# Autodesk Inventor assembly: Clutch Concept
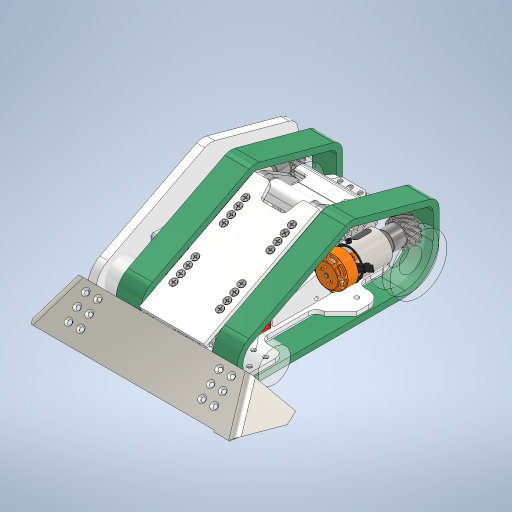
[picture p0: Inventor's stored thumbnail of the model, 512x512]
Saved by Autodesk Inventor 2023.4 (Build 274418000, 418)
## iProperties
Created: 2024-02-03
Part Number: Clutch Concept
Document SubType Name: Assembly
Designer: Nathan Cai
Mass: 1169.62 g
Surface Area: 3186.52 cm^2
Volume: 483.898 cm^3
Density: 2.41709 g/cm^3
Author: Nathan Cai
## Documents named in this file (51)
- E:\Documents\Inventor\Bleep V2\Clutch Concept.iam
- E:\Documents\Inventor\Bleep V2\Flywheel.ipt
- E:\Documents\Inventor\Bleep V2\Thrust Bearing.ipt
- E:\Documents\Inventor\Bleep V2\BB 13x19x4.ipt
- E:\Documents\Inventor\Bleep V2\Cup.ipt
- E:\Documents\Inventor\Bleep V2\1561T741_Stacked Wave Disc Spring\1561T741_Stacked Wave Disc Spring.ipt
- E:\Documents\Inventor\Bleep V2\AKK RS2205 2300KV\AKK RS2205 2300KV.iam
- E:\Documents\Inventor\Bleep V2\Nut Strip 2x1 - 4-40.ipt
- E:\Documents\Inventor\Bleep V2\BB 37mm x 30mm x 4mm.ipt
- E:\Documents\Inventor\Bleep V2\Motor Plate.ipt
- E:\Documents\Inventor\Bleep V2\Uprights.ipt
- E:\Documents\Inventor\Bleep V2\Nut Strip 4x4 - 4-40.ipt
- E:\Documents\Inventor\Bleep V2\5172T23_Metal Gear - 20 Degree Pressure Angle\5172T23_Metal Gear - 20 Degree Pressure Angle.ipt
- E:\Documents\Inventor\Bleep V2\BB .25x.5x.1875 - Flangeless.ipt
- E:\Documents\Inventor\Content Center Files\R2023\en-US\ANSI B18.3(13)\ANSI B18.3 - 4-40 UNC - 0.375(22).ipt
- E:\Documents\Inventor\Bleep V2\Lever.ipt
- E:\Documents\Inventor\Bleep V2\Servo Support.ipt
- E:\Documents\Inventor\Bleep V2\Part1\Part1.ipt
- E:\Documents\Inventor\Bleep V2\Cam - Lever.ipt
- E:\Documents\Inventor\Bleep V2\Cam - Shell.ipt
- E:\Documents\Inventor\Bleep V2\BB 3x7x3.ipt
- E:\Documents\Inventor\Bleep V2\Ramp.ipt
- E:\Documents\Inventor\Bleep V2\Lever - Copy.ipt
- E:\Documents\Inventor\Bleep V2\Brace.ipt
- E:\Documents\Inventor\Bleep V2\BB 3x7x3 - Copy.ipt
- E:\Documents\Inventor\Bleep V2\Shaft - Arms.ipt
- E:\Documents\Inventor\Bleep V2\Shaft - Flywheel C.ipt
- E:\Documents\Inventor\Bleep V2\Clutch C.ipt
- E:\Documents\Inventor\Bleep V2\9293K44_Constant-Force Spring\9293K44_Constant-Force Spring.ipt
- E:\Documents\Inventor\Bleep V2\Spring Mount.ipt
- E:\Documents\Inventor\Bleep V2\Spring Spool.ipt
- E:\Documents\Inventor\Bleep V2\Collar.ipt
- E:\Documents\Inventor\Bleep V2\Bottom Plate.ipt
- E:\Documents\Inventor\Content Center Files\R2023\en-US\ANSI B18.6.3(12)\ANSI B18.6.3 - 4-40 UNC - 0.375(15_).ipt
- E:\Documents\Inventor\Bleep V2\Crown.ipt
- E:\Documents\Inventor\Bleep V2\Front Bumper.ipt
- E:\Documents\Inventor\Content Center Files\R2023\en-US\ANSI B18.6.3(12)\ANSI B18.6.3 - 4-40 UNC - 0.3125(15_).ipt
- E:\Documents\Inventor\Content Center Files\R2023\en-US\ANSI B18.6.3(12)\ANSI B18.6.3 - 6-32 UNC - 0.375(15_).ipt
- E:\Documents\Inventor\Content Center Files\R2023\en-US\ANSI B18.2.2(06)\ANSI B18.2.2 - 6 - 32(06).ipt
- E:\Documents\Inventor\Content Center Files\R2023\en-US\ANSI B18.6.3(14)\ANSI B18.6.3 - 6-32 UNC - 0.625(6).ipt
- E:\Documents\Inventor\Bleep V2\Rack - Slot.ipt
- E:\Documents\Inventor\Bleep V2\Pin Cap - Slot.ipt
- E:\Documents\Inventor\Bleep V2\Export\STL\Lever Spacer.ipt
- E:\Documents\Inventor\Bleep V2\Ranglebox Mars-25 Assembly - Simple\Ranglebox Mars-25 Assembly - Simple.ipt
- E:\Documents\Inventor\Bleep V2\3598N291_High-Power Metal Gear\3598N291_High-Power Metal Gear.ipt
- E:\Documents\Inventor\Bleep V2\Temp Sprocket.ipt
- E:\Documents\Inventor\Bleep V2\Temp Sprocket Front.ipt
- E:\Documents\Inventor\Bleep V2\Temp Tread.ipt
- E:\Documents\Inventor\Bleep V2\Wedge.ipt
- E:\Documents\Inventor\Bleep V2\Temp Side.ipt
- E:\Documents\Inventor\Bleep V2\Tattu 4S 850mah\Tattu 850mah 4S.iam
## Components (124 placed, 50 different names)
1. Front Bumper:1 — Angle:5
2. Bottom Plate:1 — Mate:347, Flush:153, Mate:402, Mate:403, Mate:404, Mate:405, Mate:406, Mate:407, Mate:408, Mate:409, Mate:410, Mate:411, Mate:412, Mate:413, Mate:414, Mate:415, Mate:416, Mate:417, Mate:418, Mate:420, Mate:422, Mate:424, Angle:6
3. Cross Recessed Flat Countersunk Head Machine Screw - Type II - Inch 6-32 x 5/8:1
4. Crown:1 — Mate:386, Mate:387
5. Spline Socket Head Cap Screw - Inch 4-40 UNC - 0.375:9 — Mate:427, Mate:428
6. Spline Socket Head Cap Screw - Inch 4-40 UNC - 0.375:10 — Mate:429, Mate:430
7. Spline Socket Head Cap Screw - Inch 4-40 UNC - 0.375:11 — Mate:431, Mate:432
8. Spline Socket Head Cap Screw - Inch 4-40 UNC - 0.375:12 — Mate:433, Mate:434
9. Spline Socket Head Cap Screw - Inch 4-40 UNC - 0.375:13 — Mate:435, Mate:436
10. Spline Socket Head Cap Screw - Inch 4-40 UNC - 0.375:14 — Mate:437, Mate:438
11. Spline Socket Head Cap Screw - Inch 4-40 UNC - 0.375:15 — Mate:439, Mate:440
12. Spline Socket Head Cap Screw - Inch 4-40 UNC - 0.375:16 — Mate:441, Mate:442
13. Spline Socket Head Cap Screw - Inch 4-40 UNC - 0.375:17 — Mate:443, Mate:444
14. Spline Socket Head Cap Screw - Inch 4-40 UNC - 0.375:18 — Mate:445, Mate:446
15. Spline Socket Head Cap Screw - Inch 4-40 UNC - 0.375:19 — Mate:447, Mate:448
16. Spline Socket Head Cap Screw - Inch 4-40 UNC - 0.375:20 — Mate:449, Mate:450
17. Spline Socket Head Cap Screw - Inch 4-40 UNC - 0.375:21 — Mate:451, Mate:452
18. Spline Socket Head Cap Screw - Inch 4-40 UNC - 0.375:22 — Mate:453, Mate:454
19. Spline Socket Head Cap Screw - Inch 4-40 UNC - 0.375:23 — Mate:455, Mate:456
20. Spline Socket Head Cap Screw - Inch 4-40 UNC - 0.375:24 — Mate:457, Mate:458
21. Pin Cap - Slot:1 — Mate:459, Mate:460, Mate:461
22. Lever Spacer:1 — Mate:462, Mate:463
23. Ranglebox Mars-25 Assembly - Simple:1 — Mate:464, Flush:154, Angle:7
24. 3598N291_High-Power Metal Gear:1 — Mate:464, Flush:154, Tangent:2
25. Temp Sprocket:1 — Tangent:2, Angle:6, Angle:7
26. Temp Sprocket Front:1
27. Temp Tread:1
28. Temp Tread:2
29. Wedge:1
30. Temp Side:1
31. Temp Side:2
32. Ranglebox Mars-25 Assembly - Simple:2
33. 3598N291_High-Power Metal Gear:2
34. Temp Sprocket:2
35. Temp Sprocket Front:2
36. Tattu 850mah 4S:1 [sub-assembly]
37. Flywheel:1 — Mate:275, Mate:309
38. Shaft - Flywheel C:1 — Mate:306, Mate:307, Mate:308, Mate:310, Mate:311, Mate:312, Mate:313, Mate:314, Mate:315, Angle:4, Mate:319, Mate:321, Mate:324, Mate:465
39. Shaft - Arms:1 — Mate:257, Flush:118, Mate:386
40. Clutch C:1 — Mate:308, Angle:4
41. Rack - Slot:1 — Angle:1, Angle:3, Rotation/Translation:1, Mate:315, Mate:313, Mate:314, Mate:459, Mate:460, Mate:461
42. Cup:1 — Mate:26, Mate:27, Angle:1, Tangent:1
43. AKK RS2205 2300KV:1 [sub-assembly] — Mate:426
44. Motor Plate:1 — Mate:106, Mate:107, Mate:128, Mate:129, Mate:131, Mate:132, Mate:134, Mate:136, Flush:106, Mate:144, Mate:145, Mate:146, Mate:147, Mate:148, Mate:149, Mate:150, Mate:151, Mate:152, Mate:153, Mate:154, Mate:155, Mate:156, Mate:157, Mate:158, Mate:159, Flush:149, Mate:426
45. 1561T741_Stacked Wave Disc Spring:1 — Mate:311, Mate:312
46. 9293K44_Constant-Force Spring:1 — Mate:323, Mate:346
47. Spring Mount:1 — Mate:316, Flush:149, Mate:317, Mate:320, Mate:323, Mate:346, Mate:465
48. Thrust Bearing:1 — Mate:319, Mate:320, Mate:322
49. Spring Spool:1 — Mate:321, Mate:322, Mate:325
50. Collar:1 — Mate:324, Mate:325
51. Uprights:1 — Mate:128, Mate:130, Flush:103, Flush:104, Mate:133, Mate:138, Mate:141, Flush:107, Mate:168, Mate:169, Flush:108, Mate:229, Mate:230, Flush:110, Mate:257, Mate:266, Mate:267, Mate:268, Mate:269, Flush:125, Mate:317, Mate:289, Mate:347, Mate:363
52. Uprights:2 — Flush:103, Mate:132, Flush:104, Mate:135, Mate:137, Mate:139, Mate:140, Mate:191, Mate:226, Mate:228, Flush:111, Mate:263, Mate:264, Mate:270, Mate:271, Flush:124, Mate:292, Mate:362, Mate:387, Angle:5
53. Brace:1 — Mate:226, Mate:228, Flush:111, Mate:292
54. Brace:2 — Mate:229, Mate:230, Flush:110, Mate:289
55. Nut Strip 4x4 - 4-40:1 — Mate:129, Mate:130, Mate:131, Mate:133, Mate:316
56. Nut Strip 4x4 - 4-40:2 — Mate:134, Mate:135, Mate:136, Mate:137
57. 5172T23_Metal Gear - 20 Degree Pressure Angle:1 — Mate:138, Mate:141, Flush:105, Angle:3, Mate:198, Mate:199, Mate:200, Mate:201, Mate:202, Mate:203, Mate:204, Rotation/Translation:1, Flush:118, Mate:369, Mate:427, Mate:428, Mate:429, Mate:430, Mate:431, Mate:432, Mate:433, Mate:434, Mate:435, Mate:436, Mate:437, Mate:438, Mate:439, Mate:440, Mate:441, Mate:442
58. 5172T23_Metal Gear - 20 Degree Pressure Angle:2 — Mate:139, Mate:140, Flush:105, Mate:192, Mate:193, Mate:194, Mate:195, Mate:196, Mate:197, Flush:150, Mate:443, Mate:444, Mate:445, Mate:446, Mate:447, Mate:448, Mate:449, Mate:450, Mate:451, Mate:452, Mate:453, Mate:454, Mate:455, Mate:456, Mate:457, Mate:458
59. BB .25x.5x.1875 - Flangeless:1 — Flush:106, Mate:310
60. Lever:1 — Mate:168, Mate:169, Tangent:1, Mate:181, Mate:182, Mate:190, Mate:326, Mate:327
61. Lever - Copy:1
62. Part1:1 — Mate:179, Mate:180, Mate:186, Mate:187, Mate:188
63. Cam - Lever:1 — Mate:177, Mate:178, Mate:327
64. Cam - Shell:1 — Mate:177, Mate:178, Mate:179, Mate:180
65. BB 3x7x3:1 — Mate:181, Mate:182
66. BB 3x7x3:2 — Mate:462, Mate:463
67. BB 3x7x3 - Copy:1 — Mate:190, Mate:326
68. BB 13x19x4:1 — Mate:26, Mate:27
69. BB 37mm x 30mm x 4mm:1 — Mate:106, Mate:107
70. BB .25x.5x.1875 - Flangeless:2 — Mate:275, Mate:306, Mate:307, Mate:309
71. Servo Support:1 — Mate:186, Mate:187, Mate:188, Flush:108, Mate:191, Flush:153, Mate:419, Mate:421, Mate:423, Mate:425
72. Ramp:1 — Mate:204, Flush:150, Mate:369, Mate:370, Mate:371, Mate:372, Mate:373, Mate:374, Mate:375, Mate:376, Mate:377, Mate:378, Mate:379, Mate:380, Mate:381, Mate:382, Mate:383, Mate:384, Mate:385
73. Nut Strip 4x4 - 4-40:3 — Mate:192, Mate:193, Mate:194
74. Nut Strip 4x4 - 4-40:5 — Mate:199, Mate:200, Mate:201
75. Nut Strip 4x4 - 4-40:6 — Mate:198, Mate:202, Mate:203
76. Nut Strip 4x4 - 4-40:7 — Mate:195, Mate:196, Mate:197
77. Nut Strip 4x4 - 4-40:8 — Mate:266, Mate:267, Mate:363
78. Nut Strip 4x4 - 4-40:9 — Mate:263, Mate:264, Mate:362
79. Nut Strip 2x1 - 4-40:3 — Mate:270, Mate:271, Flush:124
80. Nut Strip 2x1 - 4-40:4 — Mate:268, Mate:269, Flush:125
81. Cross Recessed Flat Countersunk Head Machine Screw - Type I - Inch 4-40 x 5/16:1 — Mate:402
82. Cross Recessed Flat Countersunk Head Machine Screw - Type I - Inch 4-40 x 5/16:2 — Mate:403
83. Cross Recessed Flat Countersunk Head Machine Screw - Type I - Inch 4-40 x 5/16:3 — Mate:404
84. Cross Recessed Flat Countersunk Head Machine Screw - Type I - Inch 4-40 x 5/16:4 — Mate:405
85. Cross Recessed Flat Countersunk Head Machine Screw - Type I - Inch 4-40 x 5/16:5 — Mate:406
86. Cross Recessed Flat Countersunk Head Machine Screw - Type I - Inch 4-40 x 5/16:6 — Mate:407
87. Cross Recessed Flat Countersunk Head Machine Screw - Type I - Inch 4-40 x 5/16:7 — Mate:408
88. Cross Recessed Flat Countersunk Head Machine Screw - Type I - Inch 4-40 x 5/16:8 — Mate:409
89. Cross Recessed Flat Countersunk Head Machine Screw - Type I - Inch 4-40 x 5/16:9 — Mate:410
90. Cross Recessed Flat Countersunk Head Machine Screw - Type I - Inch 4-40 x 5/16:10 — Mate:411
91. Cross Recessed Flat Countersunk Head Machine Screw - Type I - Inch 4-40 x 5/16:11 — Mate:412
92. Cross Recessed Flat Countersunk Head Machine Screw - Type I - Inch 4-40 x 5/16:12 — Mate:413
93. Cross Recessed Flat Countersunk Head Machine Screw - Type I - Inch 6-32 x 3/8:1 — Mate:414
94. Hex Machine Screw Nut - Inch 6 - 32:1 — Mate:418, Mate:419
95. Cross Recessed Flat Countersunk Head Machine Screw - Type I - Inch 6-32 x 3/8:2 — Mate:415
96. Cross Recessed Flat Countersunk Head Machine Screw - Type I - Inch 6-32 x 3/8:3 — Mate:416
97. Cross Recessed Flat Countersunk Head Machine Screw - Type I - Inch 6-32 x 3/8:4 — Mate:417
98. Hex Machine Screw Nut - Inch 6 - 32:2 — Mate:420, Mate:421
99. Hex Machine Screw Nut - Inch 6 - 32:3 — Mate:422, Mate:423
100. Hex Machine Screw Nut - Inch 6 - 32:4 — Mate:424, Mate:425
101. Cross Recessed Flat Countersunk Head Machine Screw - Type I - Inch 4-40 x 3/8:1 — Mate:370
102. Cross Recessed Flat Countersunk Head Machine Screw - Type I - Inch 4-40 x 3/8:2 — Mate:371
103. Cross Recessed Flat Countersunk Head Machine Screw - Type I - Inch 4-40 x 3/8:3 — Mate:372
104. Cross Recessed Flat Countersunk Head Machine Screw - Type I - Inch 4-40 x 3/8:4 — Mate:373
105. Cross Recessed Flat Countersunk Head Machine Screw - Type I - Inch 4-40 x 3/8:5 — Mate:374
106. Cross Recessed Flat Countersunk Head Machine Screw - Type I - Inch 4-40 x 3/8:6 — Mate:375
107. Cross Recessed Flat Countersunk Head Machine Screw - Type I - Inch 4-40 x 3/8:7 — Mate:376
108. Cross Recessed Flat Countersunk Head Machine Screw - Type I - Inch 4-40 x 3/8:8 — Mate:377
109. Cross Recessed Flat Countersunk Head Machine Screw - Type I - Inch 4-40 x 3/8:9 — Mate:378
110. Cross Recessed Flat Countersunk Head Machine Screw - Type I - Inch 4-40 x 3/8:10 — Mate:379
111. Cross Recessed Flat Countersunk Head Machine Screw - Type I - Inch 4-40 x 3/8:11 — Mate:380
112. Cross Recessed Flat Countersunk Head Machine Screw - Type I - Inch 4-40 x 3/8:12 — Mate:381
113. Cross Recessed Flat Countersunk Head Machine Screw - Type I - Inch 4-40 x 3/8:13 — Mate:382
114. Cross Recessed Flat Countersunk Head Machine Screw - Type I - Inch 4-40 x 3/8:14 — Mate:383
115. Cross Recessed Flat Countersunk Head Machine Screw - Type I - Inch 4-40 x 3/8:15 — Mate:384
116. Cross Recessed Flat Countersunk Head Machine Screw - Type I - Inch 4-40 x 3/8:16 — Mate:385
117. Spline Socket Head Cap Screw - Inch 4-40 UNC - 0.375:1 — Mate:144, Mate:145
118. Spline Socket Head Cap Screw - Inch 4-40 UNC - 0.375:2 — Mate:146, Mate:147
119. Spline Socket Head Cap Screw - Inch 4-40 UNC - 0.375:3 — Mate:148, Mate:149
120. Spline Socket Head Cap Screw - Inch 4-40 UNC - 0.375:4 — Mate:150, Mate:151
121. Spline Socket Head Cap Screw - Inch 4-40 UNC - 0.375:5 — Mate:152, Mate:153
122. Spline Socket Head Cap Screw - Inch 4-40 UNC - 0.375:6 — Mate:154, Mate:155
123. Spline Socket Head Cap Screw - Inch 4-40 UNC - 0.375:7 — Mate:156, Mate:157
124. Spline Socket Head Cap Screw - Inch 4-40 UNC - 0.375:8 — Mate:158, Mate:159
## Relationships (219: Mate 192, Flush 16, Angle 7, Tangent 3, RelateRotateTranslate 1)
- [Mate]: Clutch C:1 ↔ BB 13x19x4:1
- [Mate]: Clutch C:1 ↔ BB 13x19x4:1
- Mate:26: Cup:1 ↔ BB 13x19x4:1
- Mate:27: Cup:1 ↔ BB 13x19x4:1
- Angle:1 (0 deg): Rack - Slot:1 ↔ Cup:1
- Mate:106: Motor Plate:1 ↔ BB 37mm x 30mm x 4mm:1
- Mate:107: Motor Plate:1 ↔ BB 37mm x 30mm x 4mm:1
- Mate:128: Motor Plate:1 ↔ Uprights:1
- Mate:129: Motor Plate:1 ↔ Nut Strip 4x4 - 4-40:1
- Mate:130: Uprights:1 ↔ Nut Strip 4x4 - 4-40:1
- Mate:131: Motor Plate:1 ↔ Nut Strip 4x4 - 4-40:1
- Flush:103: Uprights:1 ↔ Uprights:2
- Mate:132: Motor Plate:1 ↔ Uprights:2
- Flush:104: Uprights:1 ↔ Uprights:2
- Mate:133: Uprights:1 ↔ Nut Strip 4x4 - 4-40:1
- Mate:134: Motor Plate:1 ↔ Nut Strip 4x4 - 4-40:2
- Mate:135: Uprights:2 ↔ Nut Strip 4x4 - 4-40:2
- Mate:136: Motor Plate:1 ↔ Nut Strip 4x4 - 4-40:2
- Mate:137: Uprights:2 ↔ Nut Strip 4x4 - 4-40:2
- Mate:138: Uprights:1 ↔ 5172T23_Metal Gear - 20 Degree Pressure Angle:1
- Mate:139: Uprights:2 ↔ 5172T23_Metal Gear - 20 Degree Pressure Angle:2
- Mate:140: Uprights:2 ↔ 5172T23_Metal Gear - 20 Degree Pressure Angle:2
- Mate:141: Uprights:1 ↔ 5172T23_Metal Gear - 20 Degree Pressure Angle:1
- Flush:105: 5172T23_Metal Gear - 20 Degree Pressure Angle:1 ↔ 5172T23_Metal Gear - 20 Degree Pressure Angle:2
- Flush:106: Motor Plate:1 ↔ BB .25x.5x.1875 - Flangeless:1
- Mate:144: Motor Plate:1 ↔ Spline Socket Head Cap Screw - Inch 4-40 UNC - 0.375:1
- Mate:145: Motor Plate:1 ↔ Spline Socket Head Cap Screw - Inch 4-40 UNC - 0.375:1
- Mate:146: Motor Plate:1 ↔ Spline Socket Head Cap Screw - Inch 4-40 UNC - 0.375:2
- Mate:147: Motor Plate:1 ↔ Spline Socket Head Cap Screw - Inch 4-40 UNC - 0.375:2
- Mate:148: Motor Plate:1 ↔ Spline Socket Head Cap Screw - Inch 4-40 UNC - 0.375:3
- Mate:149: Motor Plate:1 ↔ Spline Socket Head Cap Screw - Inch 4-40 UNC - 0.375:3
- Mate:150: Motor Plate:1 ↔ Spline Socket Head Cap Screw - Inch 4-40 UNC - 0.375:4
- Mate:151: Motor Plate:1 ↔ Spline Socket Head Cap Screw - Inch 4-40 UNC - 0.375:4
- Mate:152: Motor Plate:1 ↔ Spline Socket Head Cap Screw - Inch 4-40 UNC - 0.375:5
- Mate:153: Motor Plate:1 ↔ Spline Socket Head Cap Screw - Inch 4-40 UNC - 0.375:5
- Mate:154: Motor Plate:1 ↔ Spline Socket Head Cap Screw - Inch 4-40 UNC - 0.375:6
- Mate:155: Motor Plate:1 ↔ Spline Socket Head Cap Screw - Inch 4-40 UNC - 0.375:6
- Mate:156: Motor Plate:1 ↔ Spline Socket Head Cap Screw - Inch 4-40 UNC - 0.375:7
- Mate:157: Motor Plate:1 ↔ Spline Socket Head Cap Screw - Inch 4-40 UNC - 0.375:7
- Mate:158: Motor Plate:1 ↔ Spline Socket Head Cap Screw - Inch 4-40 UNC - 0.375:8
- Mate:159: Motor Plate:1 ↔ Spline Socket Head Cap Screw - Inch 4-40 UNC - 0.375:8
- Flush:107: Uprights:1
- Mate:168: Uprights:1 ↔ Lever:1
- Mate:169: Uprights:1 ↔ Lever:1
- Tangent:1: Cup:1 ↔ Lever:1
- Angle:3 (0 deg): Rack - Slot:1 ↔ 5172T23_Metal Gear - 20 Degree Pressure Angle:1
- [Mate]: Uprights:2 ↔ Lever - Copy:1
- [Mate]: Uprights:2 ↔ Lever - Copy:1
- [Mate]: Lever:1 ↔ Lever - Copy:1
- Mate:177: Cam - Lever:1 ↔ Cam - Shell:1
- Mate:178: Cam - Lever:1 ↔ Cam - Shell:1
- Mate:179: Part1:1 ↔ Cam - Shell:1
- Mate:180: Part1:1 ↔ Cam - Shell:1
- Mate:181: Lever:1 ↔ BB 3x7x3:1
- Mate:182: Lever:1 ↔ BB 3x7x3:1
- [Mate]: Lever - Copy:1 ↔ BB 3x7x3:2
- [Mate]: Lever - Copy:1 ↔ BB 3x7x3:2
- Mate:186: Part1:1 ↔ Servo Support:1
- Mate:187: Part1:1 ↔ Servo Support:1
- Mate:188: Part1:1 ↔ Servo Support:1
- Flush:108: Uprights:1 ↔ Servo Support:1
- Mate:190: Lever:1 ↔ BB 3x7x3 - Copy:1
- Mate:191: Uprights:2 ↔ Servo Support:1
- Mate:192: 5172T23_Metal Gear - 20 Degree Pressure Angle:2 ↔ Nut Strip 4x4 - 4-40:3
- Mate:193: 5172T23_Metal Gear - 20 Degree Pressure Angle:2 ↔ Nut Strip 4x4 - 4-40:3
- Mate:194: 5172T23_Metal Gear - 20 Degree Pressure Angle:2 ↔ Nut Strip 4x4 - 4-40:3
- Mate:195: 5172T23_Metal Gear - 20 Degree Pressure Angle:2 ↔ Nut Strip 4x4 - 4-40:7
- Mate:196: 5172T23_Metal Gear - 20 Degree Pressure Angle:2 ↔ Nut Strip 4x4 - 4-40:7
- Mate:197: 5172T23_Metal Gear - 20 Degree Pressure Angle:2 ↔ Nut Strip 4x4 - 4-40:7
- Mate:198: 5172T23_Metal Gear - 20 Degree Pressure Angle:1 ↔ Nut Strip 4x4 - 4-40:6
- Mate:199: 5172T23_Metal Gear - 20 Degree Pressure Angle:1 ↔ Nut Strip 4x4 - 4-40:5
- Mate:200: 5172T23_Metal Gear - 20 Degree Pressure Angle:1 ↔ Nut Strip 4x4 - 4-40:5
- Mate:201: 5172T23_Metal Gear - 20 Degree Pressure Angle:1 ↔ Nut Strip 4x4 - 4-40:5
- Mate:202: 5172T23_Metal Gear - 20 Degree Pressure Angle:1 ↔ Nut Strip 4x4 - 4-40:6
- Mate:203: 5172T23_Metal Gear - 20 Degree Pressure Angle:1 ↔ Nut Strip 4x4 - 4-40:6
- Mate:204: 5172T23_Metal Gear - 20 Degree Pressure Angle:1 ↔ Ramp:1
- Flush:150: 5172T23_Metal Gear - 20 Degree Pressure Angle:2 ↔ Ramp:1
- Mate:226: Uprights:2 ↔ Brace:1
- Mate:228: Uprights:2 ↔ Brace:1
- Mate:229: Uprights:1 ↔ Brace:2
- Mate:230: Uprights:1 ↔ Brace:2
- Rotation/Translation:1 [RelateRotateTranslate] (159.5929 mm): Rack - Slot:1 ↔ 5172T23_Metal Gear - 20 Degree Pressure Angle:1
- Flush:110: Uprights:1 ↔ Brace:2
- Flush:111: Uprights:2 ↔ Brace:1
- Mate:257: Shaft - Arms:1 ↔ Uprights:1
- Flush:118 (-6.35 mm): Shaft - Arms:1 ↔ 5172T23_Metal Gear - 20 Degree Pressure Angle:1
- Mate:315 (31.75 mm): Shaft - Flywheel C:1 ↔ Rack - Slot:1
- Mate:263: Uprights:2 ↔ Nut Strip 4x4 - 4-40:9
- Mate:264: Uprights:2 ↔ Nut Strip 4x4 - 4-40:9
- Mate:266: Uprights:1 ↔ Nut Strip 4x4 - 4-40:8
- Mate:267: Uprights:1 ↔ Nut Strip 4x4 - 4-40:8
- Mate:268: Uprights:1 ↔ Nut Strip 2x1 - 4-40:4
- Mate:269: Uprights:1 ↔ Nut Strip 2x1 - 4-40:4
- Mate:270: Uprights:2 ↔ Nut Strip 2x1 - 4-40:3
- Mate:271: Uprights:2 ↔ Nut Strip 2x1 - 4-40:3
- Flush:124: Uprights:2 ↔ Nut Strip 2x1 - 4-40:3
- Flush:125: Uprights:1 ↔ Nut Strip 2x1 - 4-40:4
- Mate:275: Flywheel:1 ↔ BB .25x.5x.1875 - Flangeless:2
- Mate:289: Uprights:1 ↔ Brace:2
- Mate:292: Uprights:2 ↔ Brace:1
- Mate:306: Shaft - Flywheel C:1 ↔ BB .25x.5x.1875 - Flangeless:2
- Mate:307: Shaft - Flywheel C:1 ↔ BB .25x.5x.1875 - Flangeless:2
- Mate:308: Shaft - Flywheel C:1 ↔ Clutch C:1
- Mate:309: Flywheel:1 ↔ BB .25x.5x.1875 - Flangeless:2
- Mate:310: Shaft - Flywheel C:1 ↔ BB .25x.5x.1875 - Flangeless:1
- Mate:311: Shaft - Flywheel C:1 ↔ 1561T741_Stacked Wave Disc Spring:1
- Mate:312: Shaft - Flywheel C:1 ↔ 1561T741_Stacked Wave Disc Spring:1
- Mate:313: Shaft - Flywheel C:1 ↔ Rack - Slot:1
- Mate:314: Shaft - Flywheel C:1 ↔ Rack - Slot:1
- Angle:4 (0 deg): Shaft - Flywheel C:1 ↔ Clutch C:1
- Mate:316: Spring Mount:1 ↔ Nut Strip 4x4 - 4-40:1
- Flush:149 (2.3813 mm): Motor Plate:1 ↔ Spring Mount:1
- Mate:317: Spring Mount:1 ↔ Uprights:1
- Mate:319: Shaft - Flywheel C:1 ↔ Thrust Bearing:1
- Mate:320: Spring Mount:1 ↔ Thrust Bearing:1
- Mate:321: Shaft - Flywheel C:1 ↔ Spring Spool:1
- Mate:322: Thrust Bearing:1 ↔ Spring Spool:1
- Mate:323: 9293K44_Constant-Force Spring:1 ↔ Spring Mount:1
- Mate:324: Shaft - Flywheel C:1 ↔ Collar:1
- Mate:325: Spring Spool:1 ↔ Collar:1
- Mate:326: Lever:1 ↔ BB 3x7x3 - Copy:1
- Mate:327: Lever:1 ↔ Cam - Lever:1
- Mate:346: 9293K44_Constant-Force Spring:1 ↔ Spring Mount:1
- Mate:347: Bottom Plate:1 ↔ Uprights:1
- Flush:153 (-6.35 mm): Bottom Plate:1 ↔ Servo Support:1
- Mate:362: Uprights:2 ↔ Nut Strip 4x4 - 4-40:9
- Mate:363: Uprights:1 ↔ Nut Strip 4x4 - 4-40:8
- Mate:369: 5172T23_Metal Gear - 20 Degree Pressure Angle:1 ↔ Ramp:1
- Mate:370: Ramp:1 ↔ Cross Recessed Flat Countersunk Head Machine Screw - Type I - Inch 4-40 x 3/8:1
- Mate:371: Ramp:1 ↔ Cross Recessed Flat Countersunk Head Machine Screw - Type I - Inch 4-40 x 3/8:2
- Mate:372: Ramp:1 ↔ Cross Recessed Flat Countersunk Head Machine Screw - Type I - Inch 4-40 x 3/8:3
- Mate:373: Ramp:1 ↔ Cross Recessed Flat Countersunk Head Machine Screw - Type I - Inch 4-40 x 3/8:4
- Mate:374: Ramp:1 ↔ Cross Recessed Flat Countersunk Head Machine Screw - Type I - Inch 4-40 x 3/8:5
- Mate:375: Ramp:1 ↔ Cross Recessed Flat Countersunk Head Machine Screw - Type I - Inch 4-40 x 3/8:6
- Mate:376: Ramp:1 ↔ Cross Recessed Flat Countersunk Head Machine Screw - Type I - Inch 4-40 x 3/8:7
- Mate:377: Ramp:1 ↔ Cross Recessed Flat Countersunk Head Machine Screw - Type I - Inch 4-40 x 3/8:8
- Mate:378: Ramp:1 ↔ Cross Recessed Flat Countersunk Head Machine Screw - Type I - Inch 4-40 x 3/8:9
- Mate:379: Ramp:1 ↔ Cross Recessed Flat Countersunk Head Machine Screw - Type I - Inch 4-40 x 3/8:10
- Mate:380: Ramp:1 ↔ Cross Recessed Flat Countersunk Head Machine Screw - Type I - Inch 4-40 x 3/8:11
- Mate:381: Ramp:1 ↔ Cross Recessed Flat Countersunk Head Machine Screw - Type I - Inch 4-40 x 3/8:12
- Mate:382: Ramp:1 ↔ Cross Recessed Flat Countersunk Head Machine Screw - Type I - Inch 4-40 x 3/8:13
- Mate:383: Ramp:1 ↔ Cross Recessed Flat Countersunk Head Machine Screw - Type I - Inch 4-40 x 3/8:14
- Mate:384: Ramp:1 ↔ Cross Recessed Flat Countersunk Head Machine Screw - Type I - Inch 4-40 x 3/8:15
- Mate:385: Ramp:1 ↔ Cross Recessed Flat Countersunk Head Machine Screw - Type I - Inch 4-40 x 3/8:16
- Mate:386: Crown:1 ↔ Shaft - Arms:1
- Mate:387: Crown:1 ↔ Uprights:2
- Angle:5 (180 deg): Front Bumper:1 ↔ Uprights:2
- Mate:402: Bottom Plate:1 ↔ Cross Recessed Flat Countersunk Head Machine Screw - Type I - Inch 4-40 x 5/16:1
- Mate:403: Bottom Plate:1 ↔ Cross Recessed Flat Countersunk Head Machine Screw - Type I - Inch 4-40 x 5/16:2
- Mate:404: Bottom Plate:1 ↔ Cross Recessed Flat Countersunk Head Machine Screw - Type I - Inch 4-40 x 5/16:3
- Mate:405: Bottom Plate:1 ↔ Cross Recessed Flat Countersunk Head Machine Screw - Type I - Inch 4-40 x 5/16:4
- Mate:406: Bottom Plate:1 ↔ Cross Recessed Flat Countersunk Head Machine Screw - Type I - Inch 4-40 x 5/16:5
- Mate:407: Bottom Plate:1 ↔ Cross Recessed Flat Countersunk Head Machine Screw - Type I - Inch 4-40 x 5/16:6
- Mate:408: Bottom Plate:1 ↔ Cross Recessed Flat Countersunk Head Machine Screw - Type I - Inch 4-40 x 5/16:7
- Mate:409: Bottom Plate:1 ↔ Cross Recessed Flat Countersunk Head Machine Screw - Type I - Inch 4-40 x 5/16:8
- Mate:410: Bottom Plate:1 ↔ Cross Recessed Flat Countersunk Head Machine Screw - Type I - Inch 4-40 x 5/16:9
- Mate:411: Bottom Plate:1 ↔ Cross Recessed Flat Countersunk Head Machine Screw - Type I - Inch 4-40 x 5/16:10
- Mate:412: Bottom Plate:1 ↔ Cross Recessed Flat Countersunk Head Machine Screw - Type I - Inch 4-40 x 5/16:11
- Mate:413: Bottom Plate:1 ↔ Cross Recessed Flat Countersunk Head Machine Screw - Type I - Inch 4-40 x 5/16:12
- Mate:414: Bottom Plate:1 ↔ Cross Recessed Flat Countersunk Head Machine Screw - Type I - Inch 6-32 x 3/8:1
- Mate:415: Bottom Plate:1 ↔ Cross Recessed Flat Countersunk Head Machine Screw - Type I - Inch 6-32 x 3/8:2
- Mate:416: Bottom Plate:1 ↔ Cross Recessed Flat Countersunk Head Machine Screw - Type I - Inch 6-32 x 3/8:3
- Mate:417: Bottom Plate:1 ↔ Cross Recessed Flat Countersunk Head Machine Screw - Type I - Inch 6-32 x 3/8:4
- Mate:418: Bottom Plate:1 ↔ Hex Machine Screw Nut - Inch 6 - 32:1
- Mate:419: Servo Support:1 ↔ Hex Machine Screw Nut - Inch 6 - 32:1
- Mate:420: Bottom Plate:1 ↔ Hex Machine Screw Nut - Inch 6 - 32:2
- Mate:421: Servo Support:1 ↔ Hex Machine Screw Nut - Inch 6 - 32:2
- Mate:422: Bottom Plate:1 ↔ Hex Machine Screw Nut - Inch 6 - 32:3
- Mate:423: Servo Support:1 ↔ Hex Machine Screw Nut - Inch 6 - 32:3
- Mate:424: Bottom Plate:1 ↔ Hex Machine Screw Nut - Inch 6 - 32:4
- Mate:425: Servo Support:1 ↔ Hex Machine Screw Nut - Inch 6 - 32:4
- Mate:426: AKK RS2205 2300KV:1 ↔ Motor Plate:1
- Mate:427: Spline Socket Head Cap Screw - Inch 4-40 UNC - 0.375:9 ↔ 5172T23_Metal Gear - 20 Degree Pressure Angle:1
- Mate:428: Spline Socket Head Cap Screw - Inch 4-40 UNC - 0.375:9 ↔ 5172T23_Metal Gear - 20 Degree Pressure Angle:1
- Mate:429: Spline Socket Head Cap Screw - Inch 4-40 UNC - 0.375:10 ↔ 5172T23_Metal Gear - 20 Degree Pressure Angle:1
- Mate:430: Spline Socket Head Cap Screw - Inch 4-40 UNC - 0.375:10 ↔ 5172T23_Metal Gear - 20 Degree Pressure Angle:1
- Mate:431: Spline Socket Head Cap Screw - Inch 4-40 UNC - 0.375:11 ↔ 5172T23_Metal Gear - 20 Degree Pressure Angle:1
- Mate:432: Spline Socket Head Cap Screw - Inch 4-40 UNC - 0.375:11 ↔ 5172T23_Metal Gear - 20 Degree Pressure Angle:1
- Mate:433: Spline Socket Head Cap Screw - Inch 4-40 UNC - 0.375:12 ↔ 5172T23_Metal Gear - 20 Degree Pressure Angle:1
- Mate:434: Spline Socket Head Cap Screw - Inch 4-40 UNC - 0.375:12 ↔ 5172T23_Metal Gear - 20 Degree Pressure Angle:1
- Mate:435: Spline Socket Head Cap Screw - Inch 4-40 UNC - 0.375:13 ↔ 5172T23_Metal Gear - 20 Degree Pressure Angle:1
- Mate:436: Spline Socket Head Cap Screw - Inch 4-40 UNC - 0.375:13 ↔ 5172T23_Metal Gear - 20 Degree Pressure Angle:1
- Mate:437: Spline Socket Head Cap Screw - Inch 4-40 UNC - 0.375:14 ↔ 5172T23_Metal Gear - 20 Degree Pressure Angle:1
- Mate:438: Spline Socket Head Cap Screw - Inch 4-40 UNC - 0.375:14 ↔ 5172T23_Metal Gear - 20 Degree Pressure Angle:1
- Mate:439: Spline Socket Head Cap Screw - Inch 4-40 UNC - 0.375:15 ↔ 5172T23_Metal Gear - 20 Degree Pressure Angle:1
- Mate:440: Spline Socket Head Cap Screw - Inch 4-40 UNC - 0.375:15 ↔ 5172T23_Metal Gear - 20 Degree Pressure Angle:1
- Mate:441: Spline Socket Head Cap Screw - Inch 4-40 UNC - 0.375:16 ↔ 5172T23_Metal Gear - 20 Degree Pressure Angle:1
- Mate:442: Spline Socket Head Cap Screw - Inch 4-40 UNC - 0.375:16 ↔ 5172T23_Metal Gear - 20 Degree Pressure Angle:1
- Mate:443: Spline Socket Head Cap Screw - Inch 4-40 UNC - 0.375:17 ↔ 5172T23_Metal Gear - 20 Degree Pressure Angle:2
- Mate:444: Spline Socket Head Cap Screw - Inch 4-40 UNC - 0.375:17 ↔ 5172T23_Metal Gear - 20 Degree Pressure Angle:2
- Mate:445: Spline Socket Head Cap Screw - Inch 4-40 UNC - 0.375:18 ↔ 5172T23_Metal Gear - 20 Degree Pressure Angle:2
- Mate:446: Spline Socket Head Cap Screw - Inch 4-40 UNC - 0.375:18 ↔ 5172T23_Metal Gear - 20 Degree Pressure Angle:2
- Mate:447: Spline Socket Head Cap Screw - Inch 4-40 UNC - 0.375:19 ↔ 5172T23_Metal Gear - 20 Degree Pressure Angle:2
- Mate:448: Spline Socket Head Cap Screw - Inch 4-40 UNC - 0.375:19 ↔ 5172T23_Metal Gear - 20 Degree Pressure Angle:2
- Mate:449: Spline Socket Head Cap Screw - Inch 4-40 UNC - 0.375:20 ↔ 5172T23_Metal Gear - 20 Degree Pressure Angle:2
- Mate:450: Spline Socket Head Cap Screw - Inch 4-40 UNC - 0.375:20 ↔ 5172T23_Metal Gear - 20 Degree Pressure Angle:2
- Mate:451: Spline Socket Head Cap Screw - Inch 4-40 UNC - 0.375:21 ↔ 5172T23_Metal Gear - 20 Degree Pressure Angle:2
- Mate:452: Spline Socket Head Cap Screw - Inch 4-40 UNC - 0.375:21 ↔ 5172T23_Metal Gear - 20 Degree Pressure Angle:2
- Mate:453: Spline Socket Head Cap Screw - Inch 4-40 UNC - 0.375:22 ↔ 5172T23_Metal Gear - 20 Degree Pressure Angle:2
- Mate:454: Spline Socket Head Cap Screw - Inch 4-40 UNC - 0.375:22 ↔ 5172T23_Metal Gear - 20 Degree Pressure Angle:2
- Mate:455: Spline Socket Head Cap Screw - Inch 4-40 UNC - 0.375:23 ↔ 5172T23_Metal Gear - 20 Degree Pressure Angle:2
- Mate:456: Spline Socket Head Cap Screw - Inch 4-40 UNC - 0.375:23 ↔ 5172T23_Metal Gear - 20 Degree Pressure Angle:2
- Mate:457: Spline Socket Head Cap Screw - Inch 4-40 UNC - 0.375:24 ↔ 5172T23_Metal Gear - 20 Degree Pressure Angle:2
- Mate:458: Spline Socket Head Cap Screw - Inch 4-40 UNC - 0.375:24 ↔ 5172T23_Metal Gear - 20 Degree Pressure Angle:2
- Mate:459: Pin Cap - Slot:1 ↔ Rack - Slot:1
- Mate:460: Pin Cap - Slot:1 ↔ Rack - Slot:1
- Mate:461: Pin Cap - Slot:1 ↔ Rack - Slot:1
- Mate:462: Lever Spacer:1 ↔ BB 3x7x3:2
- Mate:463: Lever Spacer:1 ↔ BB 3x7x3:2
- Mate:464: Ranglebox Mars-25 Assembly - Simple:1 ↔ 3598N291_High-Power Metal Gear:1
- Mate:465: Shaft - Flywheel C:1 ↔ Spring Mount:1
- Flush:154: Ranglebox Mars-25 Assembly - Simple:1 ↔ 3598N291_High-Power Metal Gear:1
- Tangent:2 (1.5 mm): 3598N291_High-Power Metal Gear:1 ↔ Temp Sprocket:1
- Angle:6 (90 deg): Bottom Plate:1 ↔ Temp Sprocket:1
- Angle:7 (90 deg): Ranglebox Mars-25 Assembly - Simple:1 ↔ Temp Sprocket:1
- [Mate]: Ranglebox Mars-25 Assembly - Simple:2 ↔ 3598N291_High-Power Metal Gear:2
- [Flush]: Ranglebox Mars-25 Assembly - Simple:2 ↔ 3598N291_High-Power Metal Gear:2
- [Tangent] (1.5 mm): 3598N291_High-Power Metal Gear:2 ↔ Temp Sprocket:2
- [Angle] (90 deg): Ranglebox Mars-25 Assembly - Simple:2 ↔ Temp Sprocket:2
## Named parameters: d944_d938 = 0 mm, d945_d943 = 90 deg, d946_d941 = 1.5 mm, d947_d940 = 0 mm
